# Autodesk Inventor assembly: vehicle assembly v2
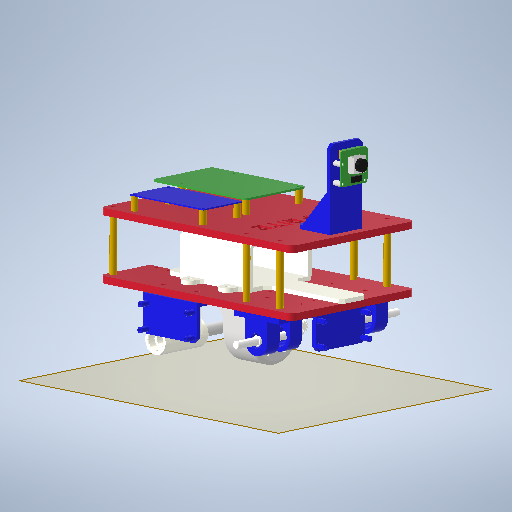
[picture p0: Inventor's stored thumbnail of the model, 512x512]
Saved by Autodesk Inventor 2025 (Build 290162010, 162A)
## iProperties
Created: 2024-06-06
Part Number: vehicle assembly v2
Document SubType Name: Assembly
Designer: david
Author: david
## Documents named in this file (28)
- F:\WRO2024FutureEngineers-Team_SPRITE_Skibidi\model\vehicle assembly v2.iam
- F:\WRO2024FutureEngineers-Team_SPRITE_Skibidi\model\base plate.ipt
- F:\WRO2024FutureEngineers-Team_SPRITE_Skibidi\model\bearing holder.ipt
- F:\WRO2024FutureEngineers-Team_SPRITE_Skibidi\model\servo motor HS-7955TG.iam
- F:\WRO2024FutureEngineers-Team_SPRITE_Skibidi\model\steering top half.ipt
- steering top half.ipt
- F:\WRO2024FutureEngineers-Team_SPRITE_Skibidi\model\dfifferential.ipt
- F:\WRO2024FutureEngineers-Team_SPRITE_Skibidi\model\front wheel.ipt
- F:\WRO2024FutureEngineers-Team_SPRITE_Skibidi\model\rear wheel 86mm.ipt
- F:\WRO2024FutureEngineers-Team_SPRITE_Skibidi\model\rear shaft.ipt
- rear shaft.ipt
- F:\WRO2024FutureEngineers-Team_SPRITE_Skibidi\model\stand M3-L10.ipt
- F:\WRO2024FutureEngineers-Team_SPRITE_Skibidi\model\top plate.ipt
- F:\WRO2024FutureEngineers-Team_SPRITE_Skibidi\model\raspberry pi.ipt
- C:\Users\limfe\Downloads\vehicle 3D model\3s lipo battery.ipt
- F:\WRO2024FutureEngineers-Team_SPRITE_Skibidi\model\ultrasonic mount.ipt
- F:\WRO2024FutureEngineers-Team_SPRITE_Skibidi\model\US-015.ipt
- F:\WRO2024FutureEngineers-Team_SPRITE_Skibidi\model\stand M3-L30.ipt
- F:\WRO2024FutureEngineers-Team_SPRITE_Skibidi\model\LM2596 Buck Converter.ipt
- F:\WRO2024FutureEngineers-Team_SPRITE_Skibidi\model\camera mount.ipt
- F:\WRO2024FutureEngineers-Team_SPRITE_Skibidi\model\raspberry pi camera.ipt
- F:\WRO2024FutureEngineers-Team_SPRITE_Skibidi\model\stub.ipt
- F:\WRO2024FutureEngineers-Team_SPRITE_Skibidi\model\steering bottom half.ipt
- F:\WRO2024FutureEngineers-Team_SPRITE_Skibidi\model\driver gear adapter v2.ipt
- F:\WRO2024FutureEngineers-Team_SPRITE_Skibidi\model\ultrasonic mount (front) v2.ipt
- F:\WRO2024FutureEngineers-Team_SPRITE_Skibidi\model\3S lipo holder v2.ipt
- F:\WRO2024FutureEngineers-Team_SPRITE_Skibidi\model\12v DC motor mount v2.ipt
- F:\WRO2024FutureEngineers-Team_SPRITE_Skibidi\model\axle-skibidi-v2.ipt
## Components (55 placed, 25 different names)
1. base plate:1 — Insert:60, Insert:61, Insert:62, Insert:63, Mate:9, Mate:10, Mate:11, Flush:6, Flush:7, Flush:8, Insert:74, Insert:75, Insert:134, Insert:135, Insert:136, Insert:137, Insert:138, Insert:139, Insert:140, Insert:141, Insert:196, Insert:197, Insert:198, Insert:199, Insert:200, Insert:201, Insert:202, Insert:203, Mate:19, Insert:208, Insert:209
2. top plate:1 — Insert:153, Insert:175, Insert:176, Insert:177, Insert:186, Insert:187, Insert:188, Insert:189, Insert:190, Insert:191
3. bearing holder:1 — Insert:134, Insert:135, Insert:143
4. bearing holder:2 — Insert:136, Insert:137
5. bearing holder:3 — Insert:140, Insert:141
6. bearing holder:4 — Insert:138, Insert:139, Insert:142
7. dfifferential:1 — Mate:16, Flush:10
8. rear shaft:1 — Insert:83, Angle:9, Insert:143, Mate:16
9. rear shaft:2 — Angle:8, Insert:142, Insert:205
10. rear wheel 86mm:1 — Insert:83, Angle:9
11. rear wheel 86mm:2 — Tangent:1, Angle:8, Insert:205
12. servo motor HS-7955TG:1 [sub-assembly] — Mate:2, Insert:20, Mate:9, Mate:10, Mate:11
13. steering top half:1 — Insert:20, Mate:14, Mate:15, Angle:12, Angle:13
14. steering bottom half:1 — Mate:14, Mate:15, Angle:12, Mate:20
15. front wheel:1
16. front wheel:2
17. stand M3-L30:2 — Insert:60, Insert:150
18. stand M3-L30:3 — Insert:63, Insert:146
19. stand M3-L30:1 — Insert:61, Insert:151
20. stand M3-L30:4 — Insert:62, Insert:148
21. stand M3-L30:9 — Insert:74, Insert:149
22. stand M3-L30:10 — Insert:75, Insert:147
23. stand M3-L10:1 — Insert:169, Insert:191
24. stand M3-L10:2 — Insert:168, Insert:189
25. stand M3-L10:3 — Insert:59
26. stand M3-L10:4 — Insert:58
27. 3s lipo battery:1 — Flush:9, Mate:18, Flush:11
28. ultrasonic mount:1 — Insert:102, Insert:103, Insert:200, Insert:201
29. ultrasonic mount:2 — Insert:106, Insert:107, Insert:198, Insert:199
30. US-015:1 — Insert:102, Insert:103
31. US-015:2 — Insert:106, Insert:107
32. US-015:3 — Insert:194, Insert:195
33. LM2596 Buck Converter:1 — Insert:112, Insert:113, Insert:169, Insert:170
34. stand M3-L10:5 — Insert:167, Insert:188
35. stand M3-L10:6 — Insert:170, Insert:190
36. stand M3-L10:7 — Insert:112
37. stand M3-L10:8 — Insert:113
38. raspberry pi:1 — Insert:58, Insert:59, Insert:167, Insert:168
39. camera mount:1 — Insert:124, Insert:125, Insert:186, Insert:187
40. raspberry pi camera:1 — Insert:120, Insert:121, Insert:122, Insert:123
41. stub:1 — Insert:123
42. stub:2 — Insert:121, Insert:124
43. stub:3 — Insert:122
44. stub:4 — Insert:120, Insert:125
45. stand M3-L10:9 — Insert:148, Insert:177
46. stand M3-L10:10 — Insert:147
47. stand M3-L10:11 — Insert:151, Insert:153
48. stand M3-L10:12 — Insert:150, Insert:175
49. stand M3-L10:13 — Insert:149
50. stand M3-L10:14 — Insert:146, Insert:176
51. driver gear adapter v2:1
52. ultrasonic mount (front) v2:1 — Insert:194, Insert:195, Insert:196, Insert:197
53. 3S lipo holder v2:1 — Insert:202, Insert:203, Mate:18, Flush:11
54. 12v DC motor mount v2:1 — Mate:19, Insert:208, Insert:209
55. axle-skibidi-v2:1 — Mate:20
## Relationships (87: Insert 65, Mate 10, Flush 6, Angle 5, Tangent 1)
- Mate:2: servo motor HS-7955TG:1
- Insert:20: servo motor HS-7955TG:1 ↔ steering top half:1
- Angle:4 (0 deg)
- Tangent:1: rear wheel 86mm:2
- Insert:58: stand M3-L10:4 ↔ raspberry pi:1
- Insert:59: stand M3-L10:3 ↔ raspberry pi:1
- Insert:60: base plate:1 ↔ stand M3-L30:2
- Insert:61: base plate:1 ↔ stand M3-L30:1
- Insert:62: base plate:1 ↔ stand M3-L30:4
- Insert:63: base plate:1 ↔ stand M3-L30:3
- Mate:9: base plate:1 ↔ servo motor HS-7955TG:1
- Mate:10: base plate:1 ↔ servo motor HS-7955TG:1
- Mate:11: base plate:1 ↔ servo motor HS-7955TG:1
- Flush:6: base plate:1
- Flush:7: base plate:1
- Flush:8: base plate:1
- Insert:74: base plate:1 ↔ stand M3-L30:9
- Insert:75: base plate:1 ↔ stand M3-L30:10
- Insert:83: rear shaft:1 ↔ rear wheel 86mm:1
- Angle:8 (180 deg): rear shaft:2 ↔ rear wheel 86mm:2
- Angle:9 (180 deg): rear shaft:1 ↔ rear wheel 86mm:1
- Insert:102: ultrasonic mount:1 ↔ US-015:1
- Insert:103: ultrasonic mount:1 ↔ US-015:1
- Insert:106: ultrasonic mount:2 ↔ US-015:2
- Insert:107: ultrasonic mount:2 ↔ US-015:2
- Insert:112: LM2596 Buck Converter:1 ↔ stand M3-L10:7
- Insert:113: LM2596 Buck Converter:1 ↔ stand M3-L10:8
- Insert:120: raspberry pi camera:1 ↔ stub:4
- Insert:121: raspberry pi camera:1 ↔ stub:2
- Insert:122: raspberry pi camera:1 ↔ stub:3
- Insert:123: raspberry pi camera:1 ↔ stub:1
- Insert:124: camera mount:1 ↔ stub:2
- Insert:125: camera mount:1 ↔ stub:4
- Insert:134: base plate:1 ↔ bearing holder:1
- Insert:135: base plate:1 ↔ bearing holder:1
- Insert:136: base plate:1 ↔ bearing holder:2
- Insert:137: base plate:1 ↔ bearing holder:2
- Insert:138: base plate:1 ↔ bearing holder:4
- Insert:139: base plate:1 ↔ bearing holder:4
- Insert:140: base plate:1 ↔ bearing holder:3
- Insert:141: base plate:1 ↔ bearing holder:3
- Insert:142: bearing holder:4 ↔ rear shaft:2
- Insert:143: bearing holder:1 ↔ rear shaft:1
- Insert:146: stand M3-L30:3 ↔ stand M3-L10:14
- Insert:147: stand M3-L30:10 ↔ stand M3-L10:10
- Insert:148: stand M3-L30:4 ↔ stand M3-L10:9
- Insert:149: stand M3-L30:9 ↔ stand M3-L10:13
- Insert:150: stand M3-L30:2 ↔ stand M3-L10:12
- Insert:151: stand M3-L30:1 ↔ stand M3-L10:11
- Insert:153: top plate:1 ↔ stand M3-L10:11
- Flush:9: 3s lipo battery:1
- Mate:14: steering top half:1 ↔ steering bottom half:1
- Mate:15: steering top half:1 ↔ steering bottom half:1
- Angle:12 (180 deg): steering top half:1 ↔ steering bottom half:1
- Angle:13 (0 deg): steering top half:1
- Insert:167: stand M3-L10:5 ↔ raspberry pi:1
- Insert:168: stand M3-L10:2 ↔ raspberry pi:1
- Insert:169: stand M3-L10:1 ↔ LM2596 Buck Converter:1
- Insert:170: LM2596 Buck Converter:1 ↔ stand M3-L10:6
- Insert:175: top plate:1 ↔ stand M3-L10:12
- Insert:176: top plate:1 ↔ stand M3-L10:14
- Insert:177: top plate:1 ↔ stand M3-L10:9
- Mate:16: dfifferential:1 ↔ rear shaft:1
- Flush:10: dfifferential:1
- Insert:186: top plate:1 ↔ camera mount:1
- Insert:187: top plate:1 ↔ camera mount:1
- Insert:188: top plate:1 ↔ stand M3-L10:5
- Insert:189: top plate:1 ↔ stand M3-L10:2
- Insert:190: top plate:1 ↔ stand M3-L10:6
- Insert:191: top plate:1 ↔ stand M3-L10:1
- Insert:194: US-015:3 ↔ ultrasonic mount (front) v2:1
- Insert:195: US-015:3 ↔ ultrasonic mount (front) v2:1
- Insert:196: base plate:1 ↔ ultrasonic mount (front) v2:1
- Insert:197: base plate:1 ↔ ultrasonic mount (front) v2:1
- Insert:198: base plate:1 ↔ ultrasonic mount:2
- Insert:199: base plate:1 ↔ ultrasonic mount:2
- Insert:200: base plate:1 ↔ ultrasonic mount:1
- Insert:201: base plate:1 ↔ ultrasonic mount:1
- Insert:202: base plate:1 ↔ 3S lipo holder v2:1
- Insert:203: base plate:1 ↔ 3S lipo holder v2:1
- Mate:18: 3s lipo battery:1 ↔ 3S lipo holder v2:1
- Flush:11: 3s lipo battery:1 ↔ 3S lipo holder v2:1
- Insert:205: rear shaft:2 ↔ rear wheel 86mm:2
- Mate:19: base plate:1 ↔ 12v DC motor mount v2:1
- Insert:208: base plate:1 ↔ 12v DC motor mount v2:1
- Insert:209: base plate:1 ↔ 12v DC motor mount v2:1
- Mate:20: steering bottom half:1 ↔ axle-skibidi-v2:1
